# Autodesk Inventor assembly: Робот RRO 2021
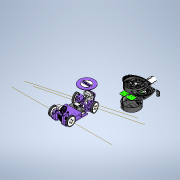
[picture p0: Inventor's stored thumbnail of the model, 180x180]
Saved by Autodesk Inventor 2020 (Build 240168000, 168)
## iProperties
Created: 2021-02-28
Part Number: Робот RRO 2021
Document SubType Name: Assembly
Designer: Антон
Author: Антон
## Documents named in this file (44)
- D:\Project\Robots\FutureEngineersViolet\3D-models\RRO 2021 Mk. IV\Робот RRO 2021 Mk. IV.iam
- D:\Project\Robots\FutureEngineersViolet\3D-models\RRO 2021 Mk. IV\Body\Основа робота.ipt
- D:\Project\Robots\FutureEngineersViolet\3D-models\RRO 2021 Mk. IV\Components\Кронштейн для двигателей серии N.ipt
- D:\Project\Robots\FutureEngineersViolet\3D-models\RRO 2021 Mk. IV\Components\Servo SG90.ipt
- D:\Project\Robots\FutureEngineersViolet\3D-models\RRO 2021 Mk. IV\Body\Основа рулевого механизма.ipt
- D:\Project\Robots\FutureEngineersViolet\3D-models\RRO 2021 Mk. IV\Components\Подшипники\Подшипник 3 8 3.ipt
- D:\Project\Robots\FutureEngineersViolet\3D-models\RRO 2021 Mk. IV\Components\Оси\Ось 3мм рулевого управления.ipt
- D:\Project\Robots\FutureEngineersViolet\3D-models\RRO 2021 Mk. IV\Body\Деталь крепления диска к поворотному механизму.ipt
- D:\Project\Robots\FutureEngineersViolet\3D-models\RRO 2021 Mk. IV\Components\Оси\Ось 3мм колеса.ipt
- D:\Project\Robots\FutureEngineersViolet\3D-models\RRO 2021 Mk. IV\Body\Деталь крепления диска к поворотному механизму_ЗЕРКАЛО1.ipt
- D:\Project\Robots\FutureEngineersViolet\3D-models\RRO 2021 Mk. IV\Components\Micro Gearmotors.ipt
- D:\Project\Robots\FutureEngineersViolet\3D-models\RRO 2021 Mk. IV\Components\Оси\Ось 2мм рулевой сервы.ipt
- D:\Project\Robots\FutureEngineersViolet\3D-models\RRO 2021 Mk. IV\Body\Поворотный рычаг для сервы.ipt
- D:\Project\Robots\FutureEngineersViolet\3D-models\RRO 2021 Mk. IV\Body\Крышка стойки подшипника 3мм.ipt
- D:\Project\Robots\FutureEngineersViolet\3D-models\RRO 2021 Mk. IV\Body\Съемная стойка сервы.ipt
- D:\Project\Robots\FutureEngineersViolet\3D-models\RRO 2021 Mk. IV\Body\Крышка поворотного кулака.ipt
- D:\Project\Robots\FutureEngineersViolet\3D-models\RRO 2021 Mk. IV\Body\Стойка подшипника 3мм.ipt
- D:\Project\Robots\FutureEngineersViolet\3D-models\RRO 2021 Mk. IV\Components\Оси\Ось 3мм задняя.ipt
- D:\Project\Robots\FutureEngineersViolet\3D-models\RRO 2021 Mk. IV\Components\Дифференциал.ipt
- D:\Project\Robots\FutureEngineersViolet\3D-models\RRO 2021 Mk. IV\Components\Подшипники\Подшипник 10 15 4.ipt
- D:\Project\Robots\FutureEngineersViolet\3D-models\RRO 2021 Mk. IV\Body\Переходник с дифференциала на ось 3мм.ipt
- D:\Project\Robots\FutureEngineersViolet\3D-models\RRO 2021 Mk. IV\Components\Оси\Ось мотора серии N.ipt
- D:\Project\Robots\FutureEngineersViolet\3D-models\RRO 2021 Mk. IV\Body\Крепление дифференциала.ipt
- D:\Project\Robots\FutureEngineersViolet\3D-models\RRO 2021 Mk. IV\Body\Деталь основы рулевого управления.ipt
- D:\Project\Robots\FutureEngineersViolet\3D-models\RRO 2021 Mk. IV\Components\Подшипники\Подшипник 3 8 4.ipt
- D:\Project\Robots\FutureEngineersViolet\3D-models\RRO 2021 Mk. IV\Components\nVision lipo battery.ipt
- D:\Project\Robots\FutureEngineersViolet\3D-models\RRO 2021 Mk. IV\Body\Рулевая тяга правая.ipt
- D:\Project\Robots\FutureEngineersViolet\3D-models\RRO 2021 Mk. IV\Body\Рулевая тяга левая.ipt
- D:\Project\Robots\FutureEngineersViolet\3D-models\RRO 2021 Mk. IV\Components\RPLIDAR A1M8\RPLIDAR A1M8.iam
- D:\Project\Robots\FutureEngineersViolet\3D-models\RRO 2021 Mk. IV\Components\Плата\Плата.iam
- D:\Project\Robots\FutureEngineersViolet\3D-models\RRO 2021 Mk. IV\Body\Крепление двигателя.ipt
- D:\Project\Robots\FutureEngineersViolet\3D-models\RRO 2021 Mk. IV\Body\Проставка для двигателя.ipt
- D:\Project\Robots\FutureEngineersViolet\3D-models\RRO 2021 Mk. IV\Body\Стойка под электроннику.ipt
- D:\Project\Robots\FutureEngineersViolet\3D-models\RRO 2021 Mk. IV\Body\Колесо D40 под планшайбу.ipt
- D:\Project\Robots\FutureEngineersViolet\3D-models\RRO 2021 Mk. IV\Components\Шина колеса D40.ipt
- D:\Project\Robots\FutureEngineersViolet\3D-models\RRO 2021 Mk. IV\Components\Планшайба D19.ipt
- D:\Project\Robots\FutureEngineersViolet\3D-models\RRO 2021 Mk. IV\Body\Крепление дифференциала_ЗЕРКАЛО.ipt
- D:\Project\Robots\FutureEngineersViolet\3D-models\RRO 2021 Mk. IV\Body\Шапка лидара.ipt
- D:\Project\Robots\FutureEngineersViolet\3D-models\RRO 2021 Mk. IV\Body\Лого ШП.ipt
- D:\Project\Robots\FutureEngineersViolet\3D-models\RRO 2021 Mk. IV\Body\Крепление камеры.ipt
- D:\Project\Robots\FutureEngineersViolet\3D-models\RRO 2021 Mk. IV\Components\Trackingcam (Applied robotics).ipt
- D:\Project\Robots\FutureEngineersViolet\3D-models\RRO 2021 Mk. IV\Body\Стойки камеры.ipt
- D:\Project\Robots\FutureEngineersViolet\3D-models\RRO 2021 Mk. IV\Body\Крепление камеры к корпусу.ipt
- D:\Project\Robots\FutureEngineersViolet\3D-models\RRO 2021 Mk. IV\Body\Ведущая шестерня дифференециала 24.ipt
## Components (72 placed, 43 different names)
1. Основа робота:1 — Жесткий:152, Жесткий:153, Жесткий:190, Жесткий:226, Жесткий:278, Жесткий:286, Жесткий:300
2. Ведущая шестерня дифференециала 24:1 — Жесткий:310, ЗубчПер:1
3. Основа рулевого механизма:1 — Жесткий:226, Жесткий:238, С поворотом:244, С поворотом:248, Жесткий:249, Жесткий:250, Жесткий:260, Жесткий:273, Жесткий:287, Жесткий:309
4. Съемная стойка сервы:1 — Жесткий:260
5. Servo SG90:2 — С поворотом:163, Жесткий:238
6. Поворотный рычаг для сервы:1 — С поворотом:163, Жесткий:259, С поворотом:250
7. Ось 2мм рулевой сервы:1 — Жесткий:259
8. Плата:1 [sub-assembly] — Жесткий:278
9. Ось 3мм задняя:2 — Жесткий:165, Жесткий:294
10. Переходник с дифференциала на ось 3мм:1 — Жесткий:165, Жесткий:171
11. Крепление двигателя:1 — Жесткий:282, Жесткий:283
12. Проставка для двигателя:1 — Жесткий:283, Жесткий:284
13. Дифференциал:1 — С поворотом:158, Жесткий:166, Жесткий:171, С поворотом:164, ЗубчПер:1
14. Переходник с дифференциала на ось 3мм:2 — Жесткий:166, Жесткий:170
15. Ось 3мм задняя:1 — Жесткий:170, Жесткий:293
16. Рулевая тяга левая:1 — С поворотом:249, С поворотом:250, С поворотом:252
17. Деталь основы рулевого управления:2 — Жесткий:248, Жесткий:250
18. Деталь крепления диска к поворотному механизму:1 — Жесткий:13, Жесткий:14, Жесткий:229, Жесткий:239, С поворотом:244, С поворотом:249
19. Крышка поворотного кулака:3 — Жесткий:239
20. Рулевая тяга правая:1 — С поворотом:251, С поворотом:252
21. Деталь основы рулевого управления:1 — Жесткий:223, Жесткий:249
22. Деталь крепления диска к поворотному механизму_ЗЕРКАЛО1:1 — Жесткий:247, Жесткий:228, Жесткий:237, Жесткий:246, С поворотом:248, С поворотом:251
23. Крышка поворотного кулака:4 — Жесткий:237
24. Trackingcam (Applied robotics):1 — Жесткий:308
25. Крепление камеры:1 — Жесткий:304, Жесткий:305, Жесткий:306, Жесткий:307, С поворотом:255
26. Крепление камеры к корпусу:1 — Жесткий:309, С поворотом:255
27. Лого ШП:1 — Жесткий:303
28. Шапка лидара:1 — Жесткий:302, Жесткий:303
29. RPLIDAR A1M8:1 [sub-assembly] — С поворотом:253, С поворотом:254, Жесткий:302
30. Стойка под электроннику:1 — Жесткий:285, Жесткий:286, С поворотом:253, С поворотом:254
31. nVision lipo battery:2 — Жесткий:285
32. Крышка стойки подшипника 3мм:1 — Жесткий:109, Жесткий:110
33. Подшипник 3*8*3:9 — Жесткий:109
34. Стойка подшипника 3мм:1 — Жесткий:110, Жесткий:153
35. Крепление дифференциала_ЗЕРКАЛО:1 — Жесткий:300, Жесткий:301
36. Подшипник 10 15 4:1 — С поворотом:158, Жесткий:301
37. Кронштейн для двигателей серии N:1 — Жесткий:174, Жесткий:284
38. Micro Gearmotors:1 — С поворотом:160, Жесткий:174
39. Ось мотора серии N:1 — С поворотом:160, Жесткий:310
40. Крепление дифференциала:2 — Жесткий:190, Жесткий:282
41. Подшипник 10 15 4:2 — С поворотом:164
42. Крышка стойки подшипника 3мм:4 — Жесткий:114, Жесткий:163
43. Подшипник 3*8*3:10 — Жесткий:163
44. Стойка подшипника 3мм:4 — Жесткий:114, Жесткий:152
45. Ось 3мм рулевого управления:3 — Жесткий:14
46. Ось 3мм колеса:1 — С поворотом:166, Жесткий:296
47. Ось 3мм рулевого управления:1 — Жесткий:13
48. Подшипник 3*8*4:1 — Жесткий:229, С поворотом:167
49. Подшипник 3*8*3:2 — Жесткий:287
50. Подшипник 3*8*3:3 — Жесткий:248
51. Ось 3мм рулевого управления:4 — Жесткий:247
52. Ось 3мм колеса:2 — С поворотом:167, Жесткий:295
53. Ось 3мм рулевого управления:5 — Жесткий:246
54. Подшипник 3*8*4:2 — Жесткий:228, С поворотом:166
55. Подшипник 3*8*3:7 — Жесткий:223
56. Подшипник 3*8*3:6 — Жесткий:273
57. Стойки камеры:2 — Жесткий:305, Жесткий:308
58. Стойки камеры:3 — Жесткий:304
59. Стойки камеры:4 — Жесткий:307
60. Стойки камеры:1 — Жесткий:306
61. Планшайба D19:3 — Жесткий:296, Жесткий:297
62. Колесо D40 под планшайбу:7 — Жесткий:292, Жесткий:297
63. Шина колеса D40:1 — Жесткий:292
64. Планшайба D19:4 — Жесткий:298, Жесткий:295
65. Колесо D40 под планшайбу:8 — Жесткий:298, Жесткий:291
66. Шина колеса D40:3 — Жесткий:291
67. Планшайба D19:2 — Жесткий:289, Жесткий:293
68. Колесо D40 под планшайбу:5 — Жесткий:288, Жесткий:289
69. Шина колеса D40:2 — Жесткий:288
70. Планшайба D19:1 — Жесткий:299, Жесткий:294
71. Колесо D40 под планшайбу:6 — Жесткий:299, Жесткий:290
72. Шина колеса D40:4 — Жесткий:290
## Relationships (75: WeldJoint 59, RevoluteJoint 15, RelateRotation 1)
- Жесткий:13 [WeldJoint]: Деталь крепления диска к поворотному механизму:1 ↔ Ось 3мм рулевого управления:1
- Жесткий:14 [WeldJoint]: Деталь крепления диска к поворотному механизму:1 ↔ Ось 3мм рулевого управления:3
- Жесткий:109 [WeldJoint] (-0.05 mm): Крышка стойки подшипника 3мм:1 ↔ Подшипник 3*8*3:9
- Жесткий:110 [WeldJoint]: Крышка стойки подшипника 3мм:1 ↔ Стойка подшипника 3мм:1
- Жесткий:114 [WeldJoint] (-0.2 mm): Крышка стойки подшипника 3мм:4 ↔ Стойка подшипника 3мм:4
- Жесткий:152 [WeldJoint]: Основа робота:1 ↔ Стойка подшипника 3мм:4
- Жесткий:153 [WeldJoint]: Основа робота:1 ↔ Стойка подшипника 3мм:1
- С поворотом:158 [RevoluteJoint] (-1 mm): Дифференциал:1 ↔ Подшипник 10 15 4:1
- Жесткий:163 [WeldJoint] (-0.05 mm): Крышка стойки подшипника 3мм:4 ↔ Подшипник 3*8*3:10
- Жесткий:165 [WeldJoint]: Ось 3мм задняя:2 ↔ Переходник с дифференциала на ось 3мм:1
- Жесткий:166 [WeldJoint]: Дифференциал:1 ↔ Переходник с дифференциала на ось 3мм:2
- Жесткий:170 [WeldJoint]: Переходник с дифференциала на ось 3мм:2 ↔ Ось 3мм задняя:1
- С поворотом:160 [RevoluteJoint]: Micro Gearmotors:1 ↔ Ось мотора серии N:1
- Жесткий:171 [WeldJoint]: Переходник с дифференциала на ось 3мм:1 ↔ Дифференциал:1
- Жесткий:174 [WeldJoint]: Кронштейн для двигателей серии N:1 ↔ Micro Gearmotors:1
- С поворотом:163 [RevoluteJoint] (2 mm): Servo SG90:2 ↔ Поворотный рычаг для сервы:1
- С поворотом:164 [RevoluteJoint] (-1 mm): Дифференциал:1 ↔ Подшипник 10 15 4:2
- Жесткий:190 [WeldJoint]: Основа робота:1 ↔ Крепление дифференциала:2
- Жесткий:223 [WeldJoint]: Деталь основы рулевого управления:1 ↔ Подшипник 3*8*3:7
- Жесткий:247 [WeldJoint]: Деталь крепления диска к поворотному механизму_ЗЕРКАЛО1:1 ↔ Ось 3мм рулевого управления:4
- Жесткий:226 [WeldJoint]: Основа робота:1 ↔ Основа рулевого механизма:1
- Жесткий:228 [WeldJoint]: Деталь крепления диска к поворотному механизму_ЗЕРКАЛО1:1 ↔ Подшипник 3*8*4:2
- С поворотом:166 [RevoluteJoint]: Ось 3мм колеса:1 ↔ Подшипник 3*8*4:2
- Жесткий:229 [WeldJoint]: Деталь крепления диска к поворотному механизму:1 ↔ Подшипник 3*8*4:1
- С поворотом:167 [RevoluteJoint]: Подшипник 3*8*4:1 ↔ Ось 3мм колеса:2
- Жесткий:237 [WeldJoint]: Деталь крепления диска к поворотному механизму_ЗЕРКАЛО1:1 ↔ Крышка поворотного кулака:4
- Жесткий:238 [WeldJoint]: Основа рулевого механизма:1 ↔ Servo SG90:2
- Жесткий:239 [WeldJoint]: Деталь крепления диска к поворотному механизму:1 ↔ Крышка поворотного кулака:3
- С поворотом:244 [RevoluteJoint] (0.8 mm): Основа рулевого механизма:1 ↔ Деталь крепления диска к поворотному механизму:1
- Жесткий:246 [WeldJoint]: Деталь крепления диска к поворотному механизму_ЗЕРКАЛО1:1 ↔ Ось 3мм рулевого управления:5
- С поворотом:248 [RevoluteJoint] (0.8 mm): Основа рулевого механизма:1 ↔ Деталь крепления диска к поворотному механизму_ЗЕРКАЛО1:1
- Жесткий:248 [WeldJoint]: Деталь основы рулевого управления:2 ↔ Подшипник 3*8*3:3
- Жесткий:249 [WeldJoint]: Основа рулевого механизма:1 ↔ Деталь основы рулевого управления:1
- Жесткий:250 [WeldJoint]: Основа рулевого механизма:1 ↔ Деталь основы рулевого управления:2
- Жесткий:259 [WeldJoint]: Поворотный рычаг для сервы:1 ↔ Ось 2мм рулевой сервы:1
- Жесткий:260 [WeldJoint]: Основа рулевого механизма:1 ↔ Съемная стойка сервы:1
- Жесткий:273 [WeldJoint]: Основа рулевого механизма:1 ↔ Подшипник 3*8*3:6
- Жесткий:278 [WeldJoint]: Основа робота:1 ↔ Плата:1
- С поворотом:249 [RevoluteJoint] (0.8 mm): Рулевая тяга левая:1 ↔ Деталь крепления диска к поворотному механизму:1
- С поворотом:250 [RevoluteJoint] (0.8 mm): Поворотный рычаг для сервы:1 ↔ Рулевая тяга левая:1
- С поворотом:251 [RevoluteJoint] (0.8 mm): Рулевая тяга правая:1 ↔ Деталь крепления диска к поворотному механизму_ЗЕРКАЛО1:1
- С поворотом:252 [RevoluteJoint] (0.8 mm): Рулевая тяга левая:1 ↔ Рулевая тяга правая:1
- Жесткий:282 [WeldJoint]: Крепление двигателя:1 ↔ Крепление дифференциала:2
- Жесткий:283 [WeldJoint]: Крепление двигателя:1 ↔ Проставка для двигателя:1
- Жесткий:284 [WeldJoint]: Проставка для двигателя:1 ↔ Кронштейн для двигателей серии N:1
- Жесткий:285 [WeldJoint]: Стойка под электроннику:1 ↔ nVision lipo battery:2
- Жесткий:286 [WeldJoint]: Основа робота:1 ↔ Стойка под электроннику:1
- Жесткий:287 [WeldJoint]: Основа рулевого механизма:1 ↔ Подшипник 3*8*3:2
- С поворотом:253 [RevoluteJoint]: RPLIDAR A1M8:1 ↔ Стойка под электроннику:1
- С поворотом:254 [RevoluteJoint]: RPLIDAR A1M8:1 ↔ Стойка под электроннику:1
- Жесткий:288 [WeldJoint]: Колесо D40 под планшайбу:5 ↔ Шина колеса D40:2
- Жесткий:289 [WeldJoint]: Планшайба D19:2 ↔ Колесо D40 под планшайбу:5
- Жесткий:298 [WeldJoint]: Планшайба D19:4 ↔ Колесо D40 под планшайбу:8
- Жесткий:299 [WeldJoint]: Планшайба D19:1 ↔ Колесо D40 под планшайбу:6
- Жесткий:290 [WeldJoint]: Колесо D40 под планшайбу:6 ↔ Шина колеса D40:4
- Жесткий:291 [WeldJoint]: Колесо D40 под планшайбу:8 ↔ Шина колеса D40:3
- Жесткий:292 [WeldJoint]: Колесо D40 под планшайбу:7 ↔ Шина колеса D40:1
- Жесткий:293 [WeldJoint]: Ось 3мм задняя:1 ↔ Планшайба D19:2
- Жесткий:294 [WeldJoint]: Ось 3мм задняя:2 ↔ Планшайба D19:1
- Жесткий:295 [WeldJoint]: Ось 3мм колеса:2 ↔ Планшайба D19:4
- Жесткий:296 [WeldJoint]: Ось 3мм колеса:1 ↔ Планшайба D19:3
- Жесткий:297 [WeldJoint]: Планшайба D19:3 ↔ Колесо D40 под планшайбу:7
- Жесткий:300 [WeldJoint]: Основа робота:1 ↔ Крепление дифференциала_ЗЕРКАЛО:1
- Жесткий:301 [WeldJoint]: Крепление дифференциала_ЗЕРКАЛО:1 ↔ Подшипник 10 15 4:1
- Жесткий:302 [WeldJoint]: Шапка лидара:1 ↔ RPLIDAR A1M8:1
- Жесткий:303 [WeldJoint]: Лого ШП:1 ↔ Шапка лидара:1
- Жесткий:304 [WeldJoint]: Крепление камеры:1 ↔ Стойки камеры:3
- Жесткий:305 [WeldJoint]: Крепление камеры:1 ↔ Стойки камеры:2
- Жесткий:306 [WeldJoint]: Крепление камеры:1 ↔ Стойки камеры:1
- Жесткий:307 [WeldJoint]: Крепление камеры:1 ↔ Стойки камеры:4
- Жесткий:308 [WeldJoint]: Trackingcam (Applied robotics):1 ↔ Стойки камеры:2
- Жесткий:309 [WeldJoint]: Основа рулевого механизма:1 ↔ Крепление камеры к корпусу:1
- С поворотом:255 [RevoluteJoint] (0.2 mm): Крепление камеры:1 ↔ Крепление камеры к корпусу:1
- Жесткий:310 [WeldJoint]: Ведущая шестерня дифференециала 24:1 ↔ Ось мотора серии N:1
- ЗубчПер:1 [RelateRotation] (0.75 ul): Ведущая шестерня дифференециала 24:1 ↔ Дифференциал:1
